# Autodesk Inventor assembly: RailWheelSys
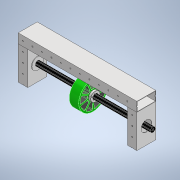
[picture p0: Inventor's stored thumbnail of the model, 180x180]
Saved by Autodesk Inventor 2022 (Build 260153000, 153)
## iProperties
Created: 2022-01-14
Part Number: RailWheelSys
Document SubType Name: Assembly
Designer: tagaz
Author: tagaz
## Documents named in this file (7)
- C:\Users\Ty Gazaway\Documents\t3-cad\CAD\2022 Parts\RailWheelSys.iam
- C:\Users\Ty Gazaway\Documents\t3-cad\CAD\2022 Parts\Generic\RailSupp.ipt
- C:\Users\Ty Gazaway\Documents\t3-cad\CAD\Bearing  for THUNDER.ipt
- C:\Users\Ty Gazaway\Documents\t3-cad\CAD\2022 Parts\Generic\railThunder.ipt
- C:\Users\Ty Gazaway\Documents\t3-cad\CAD\2022 Parts\Generic\3in Compliance wheel.ipt
- C:\Users\Ty Gazaway\Documents\t3-cad\CAD\Hex Shaft Collar.ipt
- C:\Users\Ty Gazaway\Documents\t3-cad\CAD\2022 Parts\Generic\RailSupp2.ipt
## Components (9 placed, 6 different names)
1. RailSupp:1 — Mate:1, Flush:1, Flush:2, Insert:1, Insert:2, Mate:6, Flush:5, Mate:15, Flush:6
2. RailSupp:2 — Mate:1, Flush:1, Flush:2
3. Bearing  for THUNDER:1 — Insert:1
4. Bearing  for THUNDER:2 — Insert:2, Flush:3, Mate:2, Mate:3
5. railThunder:1 — Flush:3, Mate:2, Mate:3, Mate:4, Mate:5, Mate:9, Mate:10, Mate:13, Mate:14
6. 3in Compliance wheel:1 — Mate:4, Mate:5, Mate:6, Mate:11, Mate:12
7. Hex Shaft Collar:1 — Mate:9, Mate:10, Mate:11
8. Hex Shaft Collar:2 — Mate:12, Mate:13, Mate:14
9. RailSupp2:1 — Flush:5, Mate:15, Flush:6
## Relationships (20: Mate 13, Flush 5, Insert 2)
- Mate:1 (266.7 mm): RailSupp:1 ↔ RailSupp:2
- Flush:1: RailSupp:1 ↔ RailSupp:2
- Flush:2: RailSupp:1 ↔ RailSupp:2
- Insert:1: RailSupp:1 ↔ Bearing  for THUNDER:1
- Insert:2: RailSupp:1 ↔ Bearing  for THUNDER:2
- Flush:3: Bearing  for THUNDER:2 ↔ railThunder:1
- Mate:2: Bearing  for THUNDER:2 ↔ railThunder:1
- Mate:3: Bearing  for THUNDER:2 ↔ railThunder:1
- Mate:4: railThunder:1 ↔ 3in Compliance wheel:1
- Mate:5: railThunder:1 ↔ 3in Compliance wheel:1
- Mate:6 (123.825 mm): RailSupp:1 ↔ 3in Compliance wheel:1
- Mate:9: railThunder:1 ↔ Hex Shaft Collar:1
- Mate:10: railThunder:1 ↔ Hex Shaft Collar:1
- Mate:11: 3in Compliance wheel:1 ↔ Hex Shaft Collar:1
- Mate:12: 3in Compliance wheel:1 ↔ Hex Shaft Collar:2
- Mate:13: railThunder:1 ↔ Hex Shaft Collar:2
- Mate:14: railThunder:1 ↔ Hex Shaft Collar:2
- Flush:5: RailSupp:1 ↔ RailSupp2:1
- Mate:15: RailSupp:1 ↔ RailSupp2:1
- Flush:6: RailSupp:1 ↔ RailSupp2:1
